# Autodesk Inventor assembly: Gripper
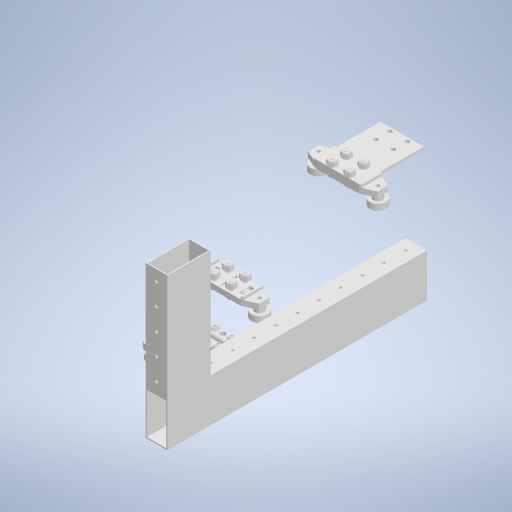
[picture p0: Inventor's stored thumbnail of the model, 512x512]
Saved by Autodesk Inventor 2023 (Build 270158000, 158)
## iProperties
Created: 2023-01-18
Part Number: Gripper
Document SubType Name: Assembly
Designer: Gabriel - T3 CAD
Author: Gabriel - T3 CAD
## Documents named in this file (5)
- C:\Users\Gabriel - T3 CAD\Documents\GitHub\t3-CAD\T3-CAD\Current Season CAD\Swerve-DriveTrain-V2.1 (LongBot)\Gripper.iam
- C:\Users\Gabriel - T3 CAD\Documents\GitHub\t3-CAD\T3-CAD\Current Season CAD\Swerve-DriveTrain-V2.1 (LongBot)\VersaFrame (Gripper-StationaryLong).ipt
- C:\Users\Gabriel - T3 CAD\Documents\GitHub\t3-CAD\T3-CAD\Current Season CAD\Swerve-DriveTrain-V2.1 (LongBot)\VersaFrame (Gripper-BaseBar).ipt
- C:\Users\Gabriel - T3 CAD\Documents\GitHub\t3-CAD\T3-CAD\Stock\ThriftyBot-Elevator\Sliding Elevator Block Assembly _1__Simplify_1.ipt
- C:\Users\Gabriel - T3 CAD\Documents\GitHub\t3-CAD\T3-CAD\Current Season CAD\Swerve-DriveTrain-V2.1 (LongBot)\Gripper Slider Connecting Plate.ipt
## Components (7 placed, 4 different names)
1. VersaFrame (Gripper-StationaryLong):1 — Mate:1, Mate:2
2. VersaFrame (Gripper-BaseBar):1 — Mate:1, Mate:2
3. Sliding Elevator Block Assembly _1__Simplify_1:1
4. Sliding Elevator Block Assembly _1__Simplify_1:2 — Mate:3, Mate:4
5. Sliding Elevator Block Assembly _1__Simplify_1:3
6. Sliding Elevator Block Assembly _1__Simplify_1:4
7. Gripper Slider Connecting Plate:1 — Mate:3, Mate:4
## Relationships (4: Mate 4)
- Mate:1: VersaFrame (Gripper-StationaryLong):1 ↔ VersaFrame (Gripper-BaseBar):1
- Mate:2: VersaFrame (Gripper-StationaryLong):1 ↔ VersaFrame (Gripper-BaseBar):1
- Mate:3: Sliding Elevator Block Assembly _1__Simplify_1:2 ↔ Gripper Slider Connecting Plate:1
- Mate:4 (0.0762 mm): Sliding Elevator Block Assembly _1__Simplify_1:2 ↔ Gripper Slider Connecting Plate:1
